# Autodesk Inventor assembly: Ensamblaje1
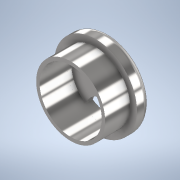
[picture p0: Inventor's stored thumbnail of the model, 180x180]
Saved by Autodesk Inventor 2020.3 (Build 243373000, 373)
## iProperties
Created: 2020-12-07
Part Number: Ensamblaje1
Document SubType Name: Assembly
Designer: codig
Author: codig
## Documents named in this file (4)
- C:\Users\codig\OneDrive\Documentos\GrabCAD\EscritorioV4\Bosquejo Pasacables\pasacables.iam
- C:\Users\codig\OneDrive\Documentos\GrabCAD\EscritorioV4\Bosquejo Pasacables\Pieza6.ipt
- C:\Users\codig\OneDrive\Documentos\GrabCAD\EscritorioV4\Bosquejo Pasacables\Pieza4.ipt
- C:\Users\codig\OneDrive\Documentos\GrabCAD\EscritorioV4\Bosquejo Pasacables\Pieza5.ipt
## Components (3 placed, 3 different names)
1. Pieza4:1 — Rígido:1
2. Pieza5:1 — Rígido:1, Insertar:1, Nivelación:1
3. Pieza6:2 — Insertar:1, Nivelación:1
## Relationships (3: WeldJoint 1, Insert 1, Flush 1)
- Rígido:1 [WeldJoint]: Pieza4:1 ↔ Pieza5:1
- Insertar:1: Pieza5:1 ↔ Pieza6:2
- Nivelación:1 [Flush]: Pieza5:1 ↔ Pieza6:2
